# Autodesk Inventor assembly: Y-Carriage_LM3037
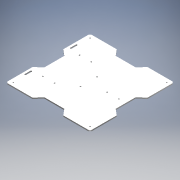
[picture p0: Inventor's stored thumbnail of the model, 180x180]
Saved by Autodesk Inventor 2020.2 (Build 242310000, 310)
## iProperties
Created: 2020-04-10
Part Number: Y-Carriage_LM3037
Document SubType Name: Assembly
Designer: rah75
Author: rah75
## Documents named in this file (6)
- C:\Users\rah75\Documents\GitHub\LETU-Maker\CAD\Autodesk Inventor\Base_3001-5999\Y-Carriage\Assemblies\Y-Carriage_LM3037.iam
- C:\Users\rah75\Documents\GitHub\LETU-Maker\CAD\Autodesk Inventor\Base_3001-5999\Y-Carriage\Fabricated_Parts\Y-Carriage_Plate_LM3033.ipt
- C:\Users\rah75\Documents\GitHub\LETU-Maker\CAD\Autodesk Inventor\Base_3001-5999\Y-Carriage\Printed_Parts\Y-Carriage_Belt_Mount_LM3035.ipt
- C:\Users\rah75\Documents\GitHub\LETU-Maker\CAD\Autodesk Inventor\Base_3001-5999\Y-Carriage\Printed_Parts\Y-Carriage_Belt_Clamp_LM3036.ipt
- C:\Users\rah75\Documents\GitHub\LETU-Maker\CAD\Autodesk Inventor\Base_3001-5999\Y-Carriage\Printed_Parts\Y-Carriage_Bearing_Mount_LM3034.ipt
- C:\Users\rah75\Documents\GitHub\LETU-Maker\CAD\Autodesk Inventor\Stock_Components_1001-2999\Fasteners\Nuts\heat_insert_m3_LM1017.ipt
## Components (13 placed, 5 different names)
1. Y-Carriage_Plate_LM3033:1 — Insert:1, Insert:2, Insert:3, Insert:10, Mate:1
2. Y-Carriage_Belt_Mount_LM3035:1 — Insert:4, Insert:5, Insert:6, Insert:7, Insert:8, Insert:9
3. Y-Carriage_Belt_Clamp_LM3036:1 — Insert:12, Mate:3
4. Y-Carriage_Bearing_Mount_LM3034:1 — Insert:2
5. Y-Carriage_Bearing_Mount_LM3034:2 — Insert:3
6. Y-Carriage_Bearing_Mount_LM3034:3 — Insert:1
7. Y-Carriage_Belt_Clamp_LM3036:2 — Insert:11, Mate:2
8. heat_insert_m3_LM1017:1 — Insert:7, Insert:12
9. heat_insert_m3_LM1017:2 — Insert:5, Mate:2
10. heat_insert_m3_LM1017:3 — Insert:6, Mate:3
11. heat_insert_m3_LM1017:4 — Insert:9, Mate:1
12. heat_insert_m3_LM1017:5 — Insert:4, Insert:11
13. heat_insert_m3_LM1017:6 — Insert:8, Insert:10
## Relationships (15: Insert 12, Mate 3)
- Insert:1: Y-Carriage_Plate_LM3033:1 ↔ Y-Carriage_Bearing_Mount_LM3034:3
- Insert:2: Y-Carriage_Plate_LM3033:1 ↔ Y-Carriage_Bearing_Mount_LM3034:1
- Insert:3: Y-Carriage_Plate_LM3033:1 ↔ Y-Carriage_Bearing_Mount_LM3034:2
- Insert:4: Y-Carriage_Belt_Mount_LM3035:1 ↔ heat_insert_m3_LM1017:5
- Insert:5: Y-Carriage_Belt_Mount_LM3035:1 ↔ heat_insert_m3_LM1017:2
- Insert:6: Y-Carriage_Belt_Mount_LM3035:1 ↔ heat_insert_m3_LM1017:3
- Insert:7: Y-Carriage_Belt_Mount_LM3035:1 ↔ heat_insert_m3_LM1017:1
- Insert:8: Y-Carriage_Belt_Mount_LM3035:1 ↔ heat_insert_m3_LM1017:6
- Insert:9: Y-Carriage_Belt_Mount_LM3035:1 ↔ heat_insert_m3_LM1017:4
- Insert:10: Y-Carriage_Plate_LM3033:1 ↔ heat_insert_m3_LM1017:6
- Mate:1: Y-Carriage_Plate_LM3033:1 ↔ heat_insert_m3_LM1017:4
- Insert:11: Y-Carriage_Belt_Clamp_LM3036:2 ↔ heat_insert_m3_LM1017:5
- Insert:12: Y-Carriage_Belt_Clamp_LM3036:1 ↔ heat_insert_m3_LM1017:1
- Mate:2: Y-Carriage_Belt_Clamp_LM3036:2 ↔ heat_insert_m3_LM1017:2
- Mate:3: Y-Carriage_Belt_Clamp_LM3036:1 ↔ heat_insert_m3_LM1017:3
